# Autodesk Inventor assembly: dovetailAssembly
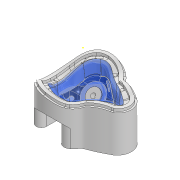
[picture p0: Inventor's stored thumbnail of the model, 180x180]
Saved by Autodesk Inventor 2021 (Build 250183000, 183)
## iProperties
Created: 2020-07-13
Part Number: dovetailAssembly
Document SubType Name: Assembly
Designer: Derm
Author: Derm
## Documents named in this file (5)
- C:\Users\Derm\n95\v7\maskBodyV4Molds\dovetailAssembly.iam
- C:\Users\Derm\n95\v7\maskBodyV4Molds\upperWithDovetails.ipt
- C:\Users\Derm\n95\v7\maskBodyV4Molds\dovetailsV2.ipt
- C:\Users\Derm\n95\v7\maskBodyV4Molds\thermoformedSupport.ipt
- C:\Users\Derm\n95\v7\maskBodyV4Molds\main.ipt
## Components (4 placed, 4 different names)
1. upperWithDovetails:1 — Flush:1, Flush:2, Flush:3, Mate:1
2. dovetailsV2:1 — Flush:1, Flush:2, Flush:3, Flush:4
3. thermoformedSupport:1 — Flush:4, Flush:5, Flush:6, Flush:7
4. main:1 — Flush:5, Flush:6, Flush:7, Mate:1
## Relationships (8: Flush 7, Mate 1)
- Flush:1: upperWithDovetails:1 ↔ dovetailsV2:1
- Flush:2: upperWithDovetails:1 ↔ dovetailsV2:1
- Flush:3: upperWithDovetails:1 ↔ dovetailsV2:1
- Flush:4: dovetailsV2:1 ↔ thermoformedSupport:1
- Flush:5: thermoformedSupport:1 ↔ main:1
- Flush:6: thermoformedSupport:1 ↔ main:1
- Flush:7: thermoformedSupport:1 ↔ main:1
- Mate:1: upperWithDovetails:1 ↔ main:1
